# Autodesk Inventor assembly: spinning thing
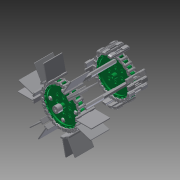
[picture p0: Inventor's stored thumbnail of the model, 180x180]
Saved by Autodesk Inventor 2014 SP1 (Build 180222100, 222)
## iProperties
Created: 2014-02-27
Part Number: spinning thing
Document SubType Name: Assembly
Designer: Ryan
Author: Ryan
## Documents named in this file (9)
- C:\Users\Ryan\Desktop\sw\toss up 4th robot\intake\spinning thing.iam
- C:\Users\Ryan\Desktop\sw\lib\Aperture VEX CAD Library\Sprockets\HS Sprockets\High strength Chain Link.ipt
- C:\Users\Ryan\Desktop\sw\lib\Aperture VEX CAD Library\Tank Tread\flap-Link.ipt
- C:\Users\Ryan\Desktop\sw\lib\Aperture VEX CAD Library\Tank Tread\flaps\Conveyor-Fin-Tall.ipt
- C:\Users\Ryan\Desktop\sw\lib\Aperture VEX CAD Library\Sprockets\green\High Strength 24-Tooth Sprocket.ipt
- C:\Users\Ryan\Desktop\sw\lib\Aperture VEX CAD Library\Spacers\SPACER-0500-0375.ipt
- C:\Users\Ryan\Desktop\sw\lib\Aperture VEX CAD Library\Standoffs\BEAM-2000.ipt
- C:\Users\Ryan\Desktop\sw\lib\Aperture VEX CAD Library\Tank Tread\Tank Tread Rubber Link.ipt
- C:\Users\Ryan\Desktop\sw\lib\Aperture VEX CAD Library\Hardware\8-32\8-32_.375.ipt
## Components (79 placed, 8 different names)
1. High Strength 24-Tooth Sprocket:1 — Mate:15, Mate:16, Mate:17, Tangent:3, Tangent:4, Mate:18, Mate:19, Mate:20, Mate:21, Mate:24, Mate:35, Mate:36
2. SPACER-0500-0375:1 — Mate:18, Mate:19
3. High Strength 24-Tooth Sprocket:2 — Mate:24, Mate:25, Mate:26, Mate:29, Tangent:5, Tangent:6, Tangent:7, Mate:30, Mate:33, Mate:34, Mate:37, Mate:38
4. High strength Chain Link:2 — Mate:13, Mate:14, Mate:15, Mate:16
5. High strength Chain Link:1 — Mate:1, Mate:2, Mate:8, Mate:13, Mate:14, Mate:17
6. Conveyor-Fin-Tall:2 — Flush:8, Mate:11, Mate:12
7. Conveyor-Fin-Tall:1 — Mate:9, Mate:10, Flush:7
8. flap-Link:1 — Mate:1, Mate:2, Mate:7, Flush:8, Mate:11, Mate:12, Tangent:3
9. flap-Link:2 — Mate:7, Mate:8, Mate:9, Mate:10, Flush:7, Tangent:4
10. High strength Chain Link:3
11. High strength Chain Link:4
12. Conveyor-Fin-Tall:3
13. Conveyor-Fin-Tall:4
14. flap-Link:3
15. flap-Link:4
16. High strength Chain Link:5
17. High strength Chain Link:6
18. Conveyor-Fin-Tall:5
19. Conveyor-Fin-Tall:6
20. flap-Link:5
21. flap-Link:6
22. High strength Chain Link:7
23. High strength Chain Link:8
24. Conveyor-Fin-Tall:7
25. Conveyor-Fin-Tall:8
26. flap-Link:7
27. flap-Link:8
28. High strength Chain Link:9
29. High strength Chain Link:10
30. Conveyor-Fin-Tall:9
31. Conveyor-Fin-Tall:10
32. flap-Link:9
33. flap-Link:10
34. High strength Chain Link:11
35. High strength Chain Link:12
36. Conveyor-Fin-Tall:11
37. Conveyor-Fin-Tall:12
38. flap-Link:11
39. flap-Link:12
40. Tank Tread Rubber Link:3 — Mate:28, Flush:31, Tangent:7
41. Tank Tread Rubber Link:2 — Mate:27, Mate:28, Flush:30, Flush:31, Tangent:6
42. Tank Tread Rubber Link:1 — Mate:27, Flush:30, Mate:29, Tangent:5, Mate:30, Mate:32
43. BEAM-2000:2 — Mate:22, Mate:23, Mate:25, Mate:26
44. BEAM-2000:1 — Mate:20, Mate:21, Mate:22, Mate:23
45. 8-32_.375:1 — Mate:35, Mate:36
46. 8-32_.375:3 — Mate:37, Mate:38
47. Tank Tread Rubber Link:4
48. Tank Tread Rubber Link:5
49. Tank Tread Rubber Link:6
50. BEAM-2000:3
51. BEAM-2000:6
52. 8-32_.375:4
53. 8-32_.375:7
54. Tank Tread Rubber Link:7
55. Tank Tread Rubber Link:8
56. Tank Tread Rubber Link:9
57. BEAM-2000:4
58. BEAM-2000:7
59. 8-32_.375:5
60. 8-32_.375:8
61. Tank Tread Rubber Link:10
62. Tank Tread Rubber Link:11
63. Tank Tread Rubber Link:12
64. BEAM-2000:5
65. BEAM-2000:8
66. 8-32_.375:6
67. 8-32_.375:9
68. High strength Chain Link:13 — Mate:32, Mate:33, Mate:34
69. High strength Chain Link:14
70. High strength Chain Link:15
71. High strength Chain Link:16
72. High strength Chain Link:17
73. High strength Chain Link:18
74. High strength Chain Link:19
75. High strength Chain Link:20
76. High strength Chain Link:21
77. High strength Chain Link:22
78. High strength Chain Link:23
79. High strength Chain Link:24
## Component patterns: (6 elements, first: High strength Chain Link:2 + High strength Chain Link:1 + Conveyor-Fin-Tall:2 + Conveyor-Fin-Tall:1 + flap-Link:1 + flap-Link:2), (4 elements, first: Tank Tread Rubber Link:3 + Tank Tread Rubber Link:2 + Tank Tread Rubber Link:1 + BEAM-2000:2 + BEAM-2000:1 + 8-32_.375:1 + 8-32_.375:3), (3 elements, first: High strength Chain Link:13), Component Pattern 5:2 (3 elements), Component Pattern 5:3 (3 elements), Component Pattern 5:4 (3 elements)
## Relationships (43: Mate 33, Flush 5, Tangent 5)
- Mate:1: High strength Chain Link:1 ↔ flap-Link:1
- Mate:2: High strength Chain Link:1 ↔ flap-Link:1
- [Flush]: High Strength 24-Tooth Sprocket:1 ↔ High strength Chain Link:1
- Mate:7: flap-Link:1 ↔ flap-Link:2
- Mate:8: High strength Chain Link:1 ↔ flap-Link:2
- Mate:9: Conveyor-Fin-Tall:1 ↔ flap-Link:2
- Mate:10: Conveyor-Fin-Tall:1 ↔ flap-Link:2
- Flush:7: Conveyor-Fin-Tall:1 ↔ flap-Link:2
- Flush:8: Conveyor-Fin-Tall:2 ↔ flap-Link:1
- Mate:11: Conveyor-Fin-Tall:2 ↔ flap-Link:1
- Mate:12: Conveyor-Fin-Tall:2 ↔ flap-Link:1
- Mate:13: High strength Chain Link:2 ↔ High strength Chain Link:1
- Mate:14: High strength Chain Link:2 ↔ High strength Chain Link:1
- Mate:15: High Strength 24-Tooth Sprocket:1 ↔ High strength Chain Link:2
- Mate:16: High Strength 24-Tooth Sprocket:1 ↔ High strength Chain Link:2
- Mate:17: High Strength 24-Tooth Sprocket:1 ↔ High strength Chain Link:1
- Tangent:3: High Strength 24-Tooth Sprocket:1 ↔ flap-Link:1
- Tangent:4: High Strength 24-Tooth Sprocket:1 ↔ flap-Link:2
- Mate:18: High Strength 24-Tooth Sprocket:1 ↔ SPACER-0500-0375:1
- Mate:19: High Strength 24-Tooth Sprocket:1 ↔ SPACER-0500-0375:1
- Mate:20: High Strength 24-Tooth Sprocket:1 ↔ BEAM-2000:1
- Mate:21: High Strength 24-Tooth Sprocket:1 ↔ BEAM-2000:1
- Mate:22: BEAM-2000:2 ↔ BEAM-2000:1
- Mate:23: BEAM-2000:2 ↔ BEAM-2000:1
- Mate:24: High Strength 24-Tooth Sprocket:1 ↔ High Strength 24-Tooth Sprocket:2
- Mate:25: High Strength 24-Tooth Sprocket:2 ↔ BEAM-2000:2
- Mate:26: High Strength 24-Tooth Sprocket:2 ↔ BEAM-2000:2
- Mate:27: Tank Tread Rubber Link:2 ↔ Tank Tread Rubber Link:1
- Mate:28: Tank Tread Rubber Link:3 ↔ Tank Tread Rubber Link:2
- Flush:30: Tank Tread Rubber Link:2 ↔ Tank Tread Rubber Link:1
- Flush:31: Tank Tread Rubber Link:3 ↔ Tank Tread Rubber Link:2
- Mate:29: High Strength 24-Tooth Sprocket:2 ↔ Tank Tread Rubber Link:1
- Tangent:5: High Strength 24-Tooth Sprocket:2 ↔ Tank Tread Rubber Link:1
- Tangent:6: High Strength 24-Tooth Sprocket:2 ↔ Tank Tread Rubber Link:2
- Tangent:7: High Strength 24-Tooth Sprocket:2 ↔ Tank Tread Rubber Link:3
- Mate:30: High Strength 24-Tooth Sprocket:2 ↔ Tank Tread Rubber Link:1
- Mate:32: Tank Tread Rubber Link:1 ↔ High strength Chain Link:13
- Mate:33: High Strength 24-Tooth Sprocket:2 ↔ High strength Chain Link:13
- Mate:34: High Strength 24-Tooth Sprocket:2 ↔ High strength Chain Link:13
- Mate:35: High Strength 24-Tooth Sprocket:1 ↔ 8-32_.375:1
- Mate:36: High Strength 24-Tooth Sprocket:1 ↔ 8-32_.375:1
- Mate:37: High Strength 24-Tooth Sprocket:2 ↔ 8-32_.375:3
- Mate:38: High Strength 24-Tooth Sprocket:2 ↔ 8-32_.375:3
